# Autodesk Inventor assembly: Track Design 9-24-19
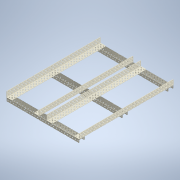
[picture p0: Inventor's stored thumbnail of the model, 180x180]
Saved by Autodesk Inventor 2020 (Build 240168000, 168)
## iProperties
Created: 2019-07-25
Part Number: Track Design 9-24-19
Document SubType Name: Assembly
Designer: Corey
Author: Corey
## Documents named in this file (3)
- C:\Users\Corey\Documents\Tower-Takeover-CAD\Parts\Dual Track.iam
- C:\Users\Corey\Documents\Tower-Takeover-CAD\Parts\Structure\90 Degree Brackets\Aluminum\Aluminum Angle 2x2x35.ipt
- C:\Users\Corey\Documents\Tower-Takeover-CAD\Parts\Structure\C-Channels\Aluminum\2-Wide\Aluminum C-Channel 1x2x1x27.ipt
## Components (7 placed, 2 different names)
1. Aluminum Angle 2x2x35:1 — Mate:1, Flush:1, Flush:2, Mate:5, Mate:6, Flush:11, Flush:12, Flush:13, Flush:14
2. Aluminum Angle 2x2x35:2 — Mate:3, Flush:8, Flush:10
3. Aluminum Angle 2x2x35:3 — Mate:2, Flush:7, Flush:9
4. Aluminum Angle 2x2x35:4 — Mate:4, Flush:3, Flush:4
5. Aluminum C-Channel 1x2x1x27:1 — Mate:6, Flush:11, Flush:12
6. Aluminum C-Channel 1x2x1x27:2 — Mate:5, Flush:13, Flush:14
7. Aluminum C-Channel 1x2x1x27:3 — Mate:1, Mate:2, Mate:3, Mate:4, Flush:1, Flush:2, Flush:3, Flush:4, Flush:7, Flush:8, Flush:9, Flush:10
## Relationships (18: Flush 12, Mate 6)
- Mate:1: Aluminum Angle 2x2x35:1 ↔ Aluminum C-Channel 1x2x1x27:3
- Mate:2: Aluminum Angle 2x2x35:3 ↔ Aluminum C-Channel 1x2x1x27:3
- Mate:3: Aluminum Angle 2x2x35:2 ↔ Aluminum C-Channel 1x2x1x27:3
- Mate:4: Aluminum Angle 2x2x35:4 ↔ Aluminum C-Channel 1x2x1x27:3
- Flush:1: Aluminum Angle 2x2x35:1 ↔ Aluminum C-Channel 1x2x1x27:3
- Flush:2: Aluminum Angle 2x2x35:1 ↔ Aluminum C-Channel 1x2x1x27:3
- Flush:3: Aluminum Angle 2x2x35:4 ↔ Aluminum C-Channel 1x2x1x27:3
- Flush:4: Aluminum Angle 2x2x35:4 ↔ Aluminum C-Channel 1x2x1x27:3
- Flush:7: Aluminum Angle 2x2x35:3 ↔ Aluminum C-Channel 1x2x1x27:3
- Flush:8: Aluminum Angle 2x2x35:2 ↔ Aluminum C-Channel 1x2x1x27:3
- Flush:9: Aluminum Angle 2x2x35:3 ↔ Aluminum C-Channel 1x2x1x27:3
- Flush:10: Aluminum Angle 2x2x35:2 ↔ Aluminum C-Channel 1x2x1x27:3
- Mate:5: Aluminum Angle 2x2x35:1 ↔ Aluminum C-Channel 1x2x1x27:2
- Mate:6: Aluminum Angle 2x2x35:1 ↔ Aluminum C-Channel 1x2x1x27:1
- Flush:11: Aluminum Angle 2x2x35:1 ↔ Aluminum C-Channel 1x2x1x27:1
- Flush:12: Aluminum Angle 2x2x35:1 ↔ Aluminum C-Channel 1x2x1x27:1
- Flush:13: Aluminum Angle 2x2x35:1 ↔ Aluminum C-Channel 1x2x1x27:2
- Flush:14: Aluminum Angle 2x2x35:1 ↔ Aluminum C-Channel 1x2x1x27:2
